# Autodesk Inventor assembly: Zlozenie_chwytak
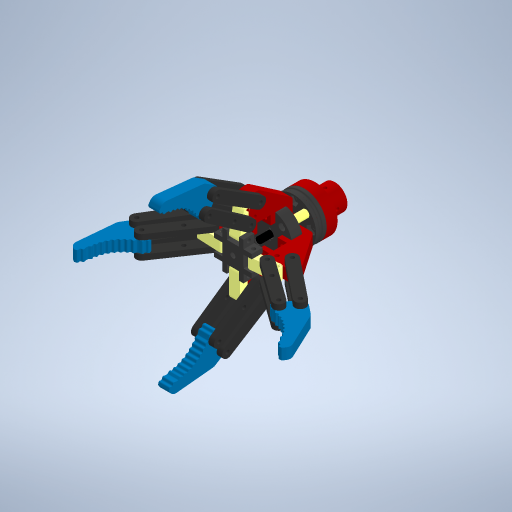
[picture p0: Inventor's stored thumbnail of the model, 512x512]
Saved by Autodesk Inventor 2023 (Build 270158000, 158)
## iProperties
Created: 2023-06-03
Part Number: Zlozenie_chwytak
Document SubType Name: Assembly
Designer: Kamil
Author: Kamil
## Documents named in this file (4)
- C:\Users\Kamil\Desktop\KONARM_2\chwytak\Zlozenie_chwytak.iam
- C:\Users\Kamil\Desktop\KONARM_2\chwytak\chwytak_core.iam
- C:\Users\Kamil\Desktop\KONARM_2\chwytak\Krzyżyk.iam
- C:\Users\Kamil\Desktop\KONARM_2\chwytak\palec.iam
## Components (6 placed, 3 different names)
1. chwytak_core:1 [sub-assembly] — Równoległe:1, Równoległe:3, Zestawiające:1, Zestawiające:5, Zestawiające:6, Zestawiające:7, Zestawiające:8, Zestawiające:9
2. Krzyżyk:1 [sub-assembly] — Równoległe:1, Równoległe:3
3. palec:1 [sub-assembly] — Równoległe:4, Zestawiające:1, Zestawiające:6
4. palec:2 [sub-assembly] — Równoległe:5, Zestawiające:7, Zestawiające:9
5. palec:3 [sub-assembly] — Równoległe:5, Zestawiające:8
6. palec:4 [sub-assembly] — Równoległe:4, Zestawiające:5
## Relationships (10: Mate 6, Flush 4)
- Równoległe:1 [Flush]: chwytak_core:1 ↔ Krzyżyk:1
- Równoległe:3 [Flush]: chwytak_core:1 ↔ Krzyżyk:1
- Równoległe:4 [Flush]: palec:1 ↔ palec:4
- Równoległe:5 [Flush]: palec:2 ↔ palec:3
- Zestawiające:1 [Mate] (0.5 mm): chwytak_core:1 ↔ palec:1
- Zestawiające:5 [Mate]: chwytak_core:1 ↔ palec:4
- Zestawiające:6 [Mate]: chwytak_core:1 ↔ palec:1
- Zestawiające:7 [Mate] (0.5 mm): chwytak_core:1 ↔ palec:2
- Zestawiające:8 [Mate]: chwytak_core:1 ↔ palec:3
- Zestawiające:9 [Mate]: chwytak_core:1 ↔ palec:2
